# Autodesk Inventor assembly: Arms
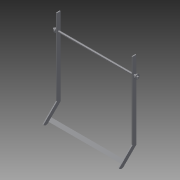
[picture p0: Inventor's stored thumbnail of the model, 180x180]
Saved by Autodesk Inventor 2013 (Build 170138000, 138)
## iProperties
Created: 2014-01-21
Part Number: Arms
Document SubType Name: Assembly
Designer: RobertB
Author: RobertB
## Documents named in this file (5)
- E:\Robotics\FRC\2014\CAD\Robot\Pickup\Arms.iam
- E:\Robotics\FRC\2014\CAD\Robot\Pickup\PickupArm.ipt
- E:\Robotics\FRC\2014\CAD\Robot\Pickup\Cloth.ipt
- E:\Robotics\FRC\2014\CAD\Robot\Pickup\SuperHexagon.ipt
- E:\Robotics\FRC\2014\CAD\Robot\Pickup\Bearing.ipt
## Components (6 placed, 4 different names)
1. PickupArm:1 — Mate:1, Flush:1, Flush:2
2. PickupArm:2 — Mate:1, Flush:1, Flush:2, Mate:4, Mate:5, Flush:4, Mate:12, Mate:13, Flush:6
3. SuperHexagon:1 — Mate:4, Mate:5, Mate:7, Mate:8, Mate:9, Mate:10, Flush:4, Flush:5
4. Bearing:1 — Mate:9, Mate:10, Mate:11
5. Bearing:2 — Mate:7, Mate:8, Mate:11, Flush:5
6. Cloth:1 — Mate:12, Mate:13, Flush:6
## Relationships (15: Mate 10, Flush 5)
- Mate:1 (508 mm): PickupArm:1 ↔ PickupArm:2
- Flush:1: PickupArm:1 ↔ PickupArm:2
- Flush:2: PickupArm:1 ↔ PickupArm:2
- Mate:4: PickupArm:2 ↔ SuperHexagon:1
- Mate:5: PickupArm:2 ↔ SuperHexagon:1
- Mate:7: SuperHexagon:1 ↔ Bearing:2
- Mate:8: SuperHexagon:1 ↔ Bearing:2
- Mate:9: SuperHexagon:1 ↔ Bearing:1
- Mate:10: SuperHexagon:1 ↔ Bearing:1
- Mate:11 (552.45 mm): Bearing:1 ↔ Bearing:2
- Flush:4 (28.575 mm): PickupArm:2 ↔ SuperHexagon:1
- Flush:5 (13.208 mm): SuperHexagon:1 ↔ Bearing:2
- Mate:12: PickupArm:2 ↔ Cloth:1
- Mate:13: PickupArm:2 ↔ Cloth:1
- Flush:6 (-25.4 mm): PickupArm:2 ↔ Cloth:1
